# Autodesk Inventor assembly: High Strength Chain Generator
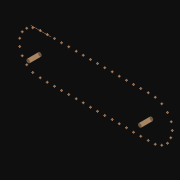
[picture p0: Inventor's stored thumbnail of the model, 180x180]
Saved by Autodesk Inventor 2021 (Build 250183000, 183)
## iProperties
RuleStatus: InUse
Created: 2020-07-07
Part Number: High Strength Chain Generator
Document SubType Name: Assembly
Designer: yuany
AfterDocOpen0: Open Form
Author: yuany
## Documents named in this file (10)
- E:\VEX Cad\Library 1.2\Motion\Chain + Tank Tread\Parametric\High Strength Chain Generator.iam
- E:\VEX Cad\Library 1.2\Motion\Chain + Tank Tread\Parametric\Workpoint Pattern.ipt
- E:\VEX Cad\Library 1.2\Motion\Chain + Tank Tread\High Strength Chain Link.ipt
- E:\VEX Cad\Library 1.2\Motion\Chain + Tank Tread\Tank Tread Traction Link.ipt
- E:\VEX Cad\Library 1.2\Motion\Chain + Tank Tread\Tread Link.ipt
- E:\VEX Cad\Library 1.2\Motion\Chain + Tank Tread\Chain Attachment Link.ipt
- E:\VEX Cad\Library 1.2\Motion\Chain + Tank Tread\Short Flap.ipt
- E:\VEX Cad\Library 1.2\Motion\Chain + Tank Tread\Medium Flap.ipt
- E:\VEX Cad\Library 1.2\Motion\Chain + Tank Tread\Tall Flap.ipt
- E:\VEX Cad\Library 1.2\Motion\Chain + Tank Tread\Parametric\Workpoint Pattern with Slack.ipt
## Components (344 placed, 8 different names)
1. Workpoint Pattern:3 — Mate:1, Mate:2, Mate:3
2. High Strength Chain Link:1 — Mate:1, Mate:2, Mate:3, Flush:1, Mate:4, Angle:1
3. High Strength Chain Link:2
4. High Strength Chain Link:3
5. High Strength Chain Link:4
6. High Strength Chain Link:5
7. High Strength Chain Link:6
8. High Strength Chain Link:7
9. High Strength Chain Link:8
10. High Strength Chain Link:9
11. High Strength Chain Link:10
12. High Strength Chain Link:11
13. High Strength Chain Link:12
14. High Strength Chain Link:13
15. High Strength Chain Link:14
16. High Strength Chain Link:15
17. High Strength Chain Link:16
18. High Strength Chain Link:17
19. High Strength Chain Link:18
20. High Strength Chain Link:19
21. High Strength Chain Link:20
22. High Strength Chain Link:21
23. High Strength Chain Link:22
24. High Strength Chain Link:23
25. High Strength Chain Link:24
26. High Strength Chain Link:25
27. High Strength Chain Link:26
28. High Strength Chain Link:27
29. High Strength Chain Link:28
30. High Strength Chain Link:29
31. High Strength Chain Link:30
32. High Strength Chain Link:31
33. High Strength Chain Link:32
34. High Strength Chain Link:33
35. High Strength Chain Link:34
36. High Strength Chain Link:35
37. High Strength Chain Link:36
38. High Strength Chain Link:37
39. High Strength Chain Link:38
40. High Strength Chain Link:39
41. High Strength Chain Link:40
42. High Strength Chain Link:41
43. High Strength Chain Link:42
44. High Strength Chain Link:43
45. High Strength Chain Link:44
46. High Strength Chain Link:45
47. High Strength Chain Link:46
48. High Strength Chain Link:47
49. High Strength Chain Link:48
50. High Strength Chain Link:49
51. Tank Tread Traction Link:1 — Flush:1, Mate:4, Angle:1, Flush:2, Mate:5, Angle:2
52. Tank Tread Traction Link:2
53. Tank Tread Traction Link:3
54. Tank Tread Traction Link:4
55. Tank Tread Traction Link:5
56. Tank Tread Traction Link:6
57. Tank Tread Traction Link:7
58. Tank Tread Traction Link:8
59. Tank Tread Traction Link:9
60. Tank Tread Traction Link:10
61. Tank Tread Traction Link:11
62. Tank Tread Traction Link:12
63. Tank Tread Traction Link:13
64. Tank Tread Traction Link:14
65. Tank Tread Traction Link:15
66. Tank Tread Traction Link:16
67. Tank Tread Traction Link:17
68. Tank Tread Traction Link:18
69. Tank Tread Traction Link:19
70. Tank Tread Traction Link:20
71. Tank Tread Traction Link:21
72. Tank Tread Traction Link:22
73. Tank Tread Traction Link:23
74. Tank Tread Traction Link:24
75. Tank Tread Traction Link:25
76. Tank Tread Traction Link:26
77. Tank Tread Traction Link:27
78. Tank Tread Traction Link:28
79. Tank Tread Traction Link:29
80. Tank Tread Traction Link:30
81. Tank Tread Traction Link:31
82. Tank Tread Traction Link:32
83. Tank Tread Traction Link:33
84. Tank Tread Traction Link:34
85. Tank Tread Traction Link:35
86. Tank Tread Traction Link:36
87. Tank Tread Traction Link:37
88. Tank Tread Traction Link:38
89. Tank Tread Traction Link:39
90. Tank Tread Traction Link:40
91. Tank Tread Traction Link:41
92. Tank Tread Traction Link:42
93. Tank Tread Traction Link:43
94. Tank Tread Traction Link:44
95. Tank Tread Traction Link:45
96. Tank Tread Traction Link:46
97. Tank Tread Traction Link:47
98. Tank Tread Traction Link:48
99. Tank Tread Traction Link:49
100. Tread Link:1 — Flush:2, Mate:5, Angle:2, Flush:3, Mate:6, Angle:3
101. Tread Link:2
102. Tread Link:3
103. Tread Link:4
104. Tread Link:5
105. Tread Link:6
106. Tread Link:7
107. Tread Link:8
108. Tread Link:9
109. Tread Link:10
110. Tread Link:11
111. Tread Link:12
112. Tread Link:13
113. Tread Link:14
114. Tread Link:15
115. Tread Link:16
116. Tread Link:17
117. Tread Link:18
118. Tread Link:19
119. Tread Link:20
120. Tread Link:21
121. Tread Link:22
122. Tread Link:23
123. Tread Link:24
124. Tread Link:25
125. Tread Link:26
126. Tread Link:27
127. Tread Link:28
128. Tread Link:29
129. Tread Link:30
130. Tread Link:31
131. Tread Link:32
132. Tread Link:33
133. Tread Link:34
134. Tread Link:35
135. Tread Link:36
136. Tread Link:37
137. Tread Link:38
138. Tread Link:39
139. Tread Link:40
140. Tread Link:41
141. Tread Link:42
142. Tread Link:43
143. Tread Link:44
144. Tread Link:45
145. Tread Link:46
146. Tread Link:47
147. Tread Link:48
148. Tread Link:49
149. Chain Attachment Link:1 — Flush:3, Mate:6, Angle:3
150. Chain Attachment Link:2
151. Chain Attachment Link:3
152. Chain Attachment Link:4
153. Chain Attachment Link:5
154. Chain Attachment Link:6
155. Chain Attachment Link:7
156. Chain Attachment Link:8
157. Chain Attachment Link:9
158. Chain Attachment Link:10
159. Chain Attachment Link:11
160. Chain Attachment Link:12
161. Chain Attachment Link:13
162. Chain Attachment Link:14
163. Chain Attachment Link:15
164. Chain Attachment Link:16
165. Chain Attachment Link:17
166. Chain Attachment Link:18
167. Chain Attachment Link:19
168. Chain Attachment Link:20
169. Chain Attachment Link:21
170. Chain Attachment Link:22
171. Chain Attachment Link:23
172. Chain Attachment Link:24
173. Chain Attachment Link:25
174. Chain Attachment Link:26
175. Chain Attachment Link:27
176. Chain Attachment Link:28
177. Chain Attachment Link:29
178. Chain Attachment Link:30
179. Chain Attachment Link:31
180. Chain Attachment Link:32
181. Chain Attachment Link:33
182. Chain Attachment Link:34
183. Chain Attachment Link:35
184. Chain Attachment Link:36
185. Chain Attachment Link:37
186. Chain Attachment Link:38
187. Chain Attachment Link:39
188. Chain Attachment Link:40
189. Chain Attachment Link:41
190. Chain Attachment Link:42
191. Chain Attachment Link:43
192. Chain Attachment Link:44
193. Chain Attachment Link:45
194. Chain Attachment Link:46
195. Chain Attachment Link:47
196. Chain Attachment Link:48
197. Chain Attachment Link:49
198. Short Flap:1 [sub-assembly]
199. Short Flap:2 [sub-assembly]
200. Short Flap:3 [sub-assembly]
201. Short Flap:4 [sub-assembly]
202. Short Flap:5 [sub-assembly]
203. Short Flap:6 [sub-assembly]
204. Short Flap:7 [sub-assembly]
205. Short Flap:8 [sub-assembly]
206. Short Flap:9 [sub-assembly]
207. Short Flap:10 [sub-assembly]
208. Short Flap:11 [sub-assembly]
209. Short Flap:12 [sub-assembly]
210. Short Flap:13 [sub-assembly]
211. Short Flap:14 [sub-assembly]
212. Short Flap:15 [sub-assembly]
213. Short Flap:16 [sub-assembly]
214. Short Flap:17 [sub-assembly]
215. Short Flap:18 [sub-assembly]
216. Short Flap:19 [sub-assembly]
217. Short Flap:20 [sub-assembly]
218. Short Flap:21 [sub-assembly]
219. Short Flap:22 [sub-assembly]
220. Short Flap:23 [sub-assembly]
221. Short Flap:24 [sub-assembly]
222. Short Flap:25 [sub-assembly]
223. Short Flap:26 [sub-assembly]
224. Short Flap:27 [sub-assembly]
225. Short Flap:28 [sub-assembly]
226. Short Flap:29 [sub-assembly]
227. Short Flap:30 [sub-assembly]
228. Short Flap:31 [sub-assembly]
229. Short Flap:32 [sub-assembly]
230. Short Flap:33 [sub-assembly]
231. Short Flap:34 [sub-assembly]
232. Short Flap:35 [sub-assembly]
233. Short Flap:36 [sub-assembly]
234. Short Flap:37 [sub-assembly]
235. Short Flap:38 [sub-assembly]
236. Short Flap:39 [sub-assembly]
237. Short Flap:40 [sub-assembly]
238. Short Flap:41 [sub-assembly]
239. Short Flap:42 [sub-assembly]
240. Short Flap:43 [sub-assembly]
241. Short Flap:44 [sub-assembly]
242. Short Flap:45
243. Short Flap:46
244. Short Flap:47
245. Short Flap:48
246. Short Flap:49
247. Medium Flap:1 [sub-assembly]
248. Medium Flap:2 [sub-assembly]
249. Medium Flap:3 [sub-assembly]
250. Medium Flap:4 [sub-assembly]
251. Medium Flap:5 [sub-assembly]
252. Medium Flap:6 [sub-assembly]
253. Medium Flap:7 [sub-assembly]
254. Medium Flap:8 [sub-assembly]
255. Medium Flap:9 [sub-assembly]
256. Medium Flap:10 [sub-assembly]
257. Medium Flap:11 [sub-assembly]
258. Medium Flap:12 [sub-assembly]
259. Medium Flap:13 [sub-assembly]
260. Medium Flap:14 [sub-assembly]
261. Medium Flap:15 [sub-assembly]
262. Medium Flap:16 [sub-assembly]
263. Medium Flap:17 [sub-assembly]
264. Medium Flap:18 [sub-assembly]
265. Medium Flap:19 [sub-assembly]
266. Medium Flap:20 [sub-assembly]
267. Medium Flap:21 [sub-assembly]
268. Medium Flap:22 [sub-assembly]
269. Medium Flap:23 [sub-assembly]
270. Medium Flap:24 [sub-assembly]
271. Medium Flap:25 [sub-assembly]
272. Medium Flap:26 [sub-assembly]
273. Medium Flap:27 [sub-assembly]
274. Medium Flap:28 [sub-assembly]
275. Medium Flap:29 [sub-assembly]
276. Medium Flap:30 [sub-assembly]
277. Medium Flap:31 [sub-assembly]
278. Medium Flap:32 [sub-assembly]
279. Medium Flap:33 [sub-assembly]
280. Medium Flap:34 [sub-assembly]
281. Medium Flap:35 [sub-assembly]
282. Medium Flap:36 [sub-assembly]
283. Medium Flap:37 [sub-assembly]
284. Medium Flap:38 [sub-assembly]
285. Medium Flap:39 [sub-assembly]
286. Medium Flap:40 [sub-assembly]
287. Medium Flap:41 [sub-assembly]
288. Medium Flap:42 [sub-assembly]
289. Medium Flap:43 [sub-assembly]
290. Medium Flap:44 [sub-assembly]
291. Medium Flap:45
292. Medium Flap:46
293. Medium Flap:47
294. Medium Flap:48
295. Medium Flap:49
296. Tall Flap:1 [sub-assembly]
297. Tall Flap:2 [sub-assembly]
298. Tall Flap:3 [sub-assembly]
299. Tall Flap:4 [sub-assembly]
300. Tall Flap:5 [sub-assembly]
301. Tall Flap:6 [sub-assembly]
302. Tall Flap:7 [sub-assembly]
303. Tall Flap:8 [sub-assembly]
304. Tall Flap:9 [sub-assembly]
305. Tall Flap:10 [sub-assembly]
306. Tall Flap:11 [sub-assembly]
307. Tall Flap:12 [sub-assembly]
308. Tall Flap:13 [sub-assembly]
309. Tall Flap:14 [sub-assembly]
310. Tall Flap:15 [sub-assembly]
311. Tall Flap:16 [sub-assembly]
312. Tall Flap:17 [sub-assembly]
313. Tall Flap:18 [sub-assembly]
314. Tall Flap:19 [sub-assembly]
315. Tall Flap:20 [sub-assembly]
316. Tall Flap:21 [sub-assembly]
317. Tall Flap:22 [sub-assembly]
318. Tall Flap:23 [sub-assembly]
319. Tall Flap:24 [sub-assembly]
320. Tall Flap:25 [sub-assembly]
321. Tall Flap:26 [sub-assembly]
322. Tall Flap:27 [sub-assembly]
323. Tall Flap:28 [sub-assembly]
324. Tall Flap:29 [sub-assembly]
325. Tall Flap:30 [sub-assembly]
326. Tall Flap:31 [sub-assembly]
327. Tall Flap:32 [sub-assembly]
328. Tall Flap:33 [sub-assembly]
329. Tall Flap:34 [sub-assembly]
330. Tall Flap:35 [sub-assembly]
331. Tall Flap:36 [sub-assembly]
332. Tall Flap:37 [sub-assembly]
333. Tall Flap:38 [sub-assembly]
334. Tall Flap:39 [sub-assembly]
335. Tall Flap:40 [sub-assembly]
336. Tall Flap:41 [sub-assembly]
337. Tall Flap:42 [sub-assembly]
338. Tall Flap:43 [sub-assembly]
339. Tall Flap:44 [sub-assembly]
340. Tall Flap:45
341. Tall Flap:46
342. Tall Flap:47
343. Tall Flap:48
344. Tall Flap:49
## Component patterns: Chain (49 elements), Traction (49 elements), Tread (49 elements), Chain Attachment (49 elements), Short Flaps (49 elements), Medium Flaps (49 elements), Tall Flaps (49 elements)
## Relationships (12: Mate 6, Flush 3, Angle 3)
- Mate:1: Workpoint Pattern:3 ↔ High Strength Chain Link:1
- Mate:2 (11.938 mm): Workpoint Pattern:3 ↔ High Strength Chain Link:1
- Mate:3: Workpoint Pattern:3 ↔ High Strength Chain Link:1
- Flush:1: High Strength Chain Link:1 ↔ Tank Tread Traction Link:1
- Mate:4: High Strength Chain Link:1 ↔ Tank Tread Traction Link:1
- Angle:1 (180 deg): High Strength Chain Link:1 ↔ Tank Tread Traction Link:1
- Flush:2: Tank Tread Traction Link:1 ↔ Tread Link:1
- Mate:5: Tank Tread Traction Link:1 ↔ Tread Link:1
- Angle:2 (0 deg): Tank Tread Traction Link:1 ↔ Tread Link:1
- Flush:3: Tread Link:1 ↔ Chain Attachment Link:1
- Mate:6: Tread Link:1 ↔ Chain Attachment Link:1
- Angle:3 (0 deg): Tread Link:1 ↔ Chain Attachment Link:1
## Named parameters: Center_Distance = 152.4 mm, Sprocket1 = 56.388 mm, Sprocket2 = 56.388 mm, CenterDistance = 152.4 mm, d5_1 = 126.66116 mm, d6_1 = 126.66116 mm, d7_1 = 84.45407 mm, d8_1 = 123.17453 mm
